# Autodesk Inventor assembly: launcher.mainAssembly
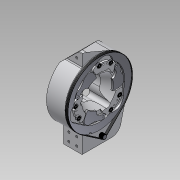
[picture p0: Inventor's stored thumbnail of the model, 180x180]
Saved by Autodesk Inventor 2011 (Build 150239000, 239)
## iProperties
Created: 2011-02-22
Part Number: launcher.mainAssembly
Document SubType Name: Assembly
Designer: Casey
Author: Casey
## Documents named in this file (8)
- C:\Users\Casey\Documents\My Dropbox\RockSAT-X 2011 RexSAT\capsule-launcher.design\Launcher\launcher.mainAssembly.iam
- C:\Users\Casey\Documents\My Dropbox\RockSAT-X 2011 RexSAT\capsule-launcher.design\Launcher\launcher.housing.ipt
- C:\Users\Casey\Documents\My Dropbox\RockSAT-X 2011 RexSAT\capsule-launcher.design\Capsule\capsule.final.assembly.iam
- C:\Users\Casey\Documents\My Dropbox\RockSAT-X 2011 RexSAT\capsule-launcher.design\Launcher\3x8x4_bearing.ipt
- C:\Users\Casey\Documents\My Dropbox\RockSAT-X 2011 RexSAT\capsule-launcher.design\Launcher\launcher.cap.ipt
- C:\Users\Casey\Documents\My Dropbox\RockSAT-X 2011 RexSAT\capsule-launcher.design\Launcher\launcher.cam.ipt
- C:\Users\Casey\Documents\My Dropbox\RockSAT-X 2011 RexSAT\capsule-launcher.design\Launcher\launcher.latch.ipt
- C:\Users\Casey\Documents\My Dropbox\RockSAT-X 2011 RexSAT\capsule-launcher.design\Launcher\launcher.mainAssembly\Design Accelerator\Synchronous Belts Transmission2.iam
## Components (17 placed, 7 different names)
1. launcher.housing:1 — Mate:7, Tangent:5, Mate:8, Mate:9, Mate:10, Mate:11, Mate:12, Mate:13, Flush:5, Mate:14, Mate:15, Mate:16, Flush:7, Mate:17, Mate:18, Mate:19, Mate:24, Mate:25, Mate:26
2. capsule.final.assembly:1 [sub-assembly] — Mate:7, Tangent:5
3. 3x8x4_bearing:1 — Mate:13, Flush:2, Flush:3
4. 3x8x4_bearing:2 — Mate:12, Flush:2, Flush:4
5. 3x8x4_bearing:3 — Mate:11, Flush:4, Flush:6
6. 3x8x4_bearing:4 — Mate:10, Flush:6
7. 3x8x4_bearing:5 — Mate:9, Flush:1, Flush:5
8. 3x8x4_bearing:6 — Mate:8, Flush:1, Flush:3
9. 3x8x4_bearing:7 — Mate:14, Flush:7, Flush:8
10. 3x8x4_bearing:8 — Mate:15, Flush:9
11. 3x8x4_bearing:9 — Mate:16, Flush:8, Flush:9, Mate:23
12. launcher.cap:1 — Mate:17, Mate:18, Mate:19
13. launcher.cam:1 — Mate:25, Mate:26
14. Synchronous Belts Transmission:1 [sub-assembly]
15. launcher.latch:1 — Mate:23, Mate:24
16. launcher.latch:2
17. launcher.latch:3
## Component patterns: (3 elements, first: launcher.latch:1)
## Relationships (27: Mate 17, Flush 9, Tangent 1)
- Mate:7: launcher.housing:1 ↔ capsule.final.assembly:1
- Tangent:5: launcher.housing:1 ↔ capsule.final.assembly:1
- Mate:8: launcher.housing:1 ↔ 3x8x4_bearing:6
- Mate:9: launcher.housing:1 ↔ 3x8x4_bearing:5
- Mate:10: launcher.housing:1 ↔ 3x8x4_bearing:4
- Mate:11: launcher.housing:1 ↔ 3x8x4_bearing:3
- Mate:12: launcher.housing:1 ↔ 3x8x4_bearing:2
- Mate:13: launcher.housing:1 ↔ 3x8x4_bearing:1
- Flush:1: 3x8x4_bearing:5 ↔ 3x8x4_bearing:6
- Flush:2: 3x8x4_bearing:1 ↔ 3x8x4_bearing:2
- Flush:3: 3x8x4_bearing:1 ↔ 3x8x4_bearing:6
- Flush:4: 3x8x4_bearing:2 ↔ 3x8x4_bearing:3
- Flush:5: launcher.housing:1 ↔ 3x8x4_bearing:5
- Flush:6: 3x8x4_bearing:3 ↔ 3x8x4_bearing:4
- Mate:14: launcher.housing:1 ↔ 3x8x4_bearing:7
- Mate:15: launcher.housing:1 ↔ 3x8x4_bearing:8
- Mate:16: launcher.housing:1 ↔ 3x8x4_bearing:9
- Flush:7: launcher.housing:1 ↔ 3x8x4_bearing:7
- Flush:8: 3x8x4_bearing:7 ↔ 3x8x4_bearing:9
- Flush:9: 3x8x4_bearing:8 ↔ 3x8x4_bearing:9
- Mate:17: launcher.housing:1 ↔ launcher.cap:1
- Mate:18: launcher.housing:1 ↔ launcher.cap:1
- Mate:19: launcher.housing:1 ↔ launcher.cap:1
- Mate:23: 3x8x4_bearing:9 ↔ launcher.latch:1
- Mate:24: launcher.housing:1 ↔ launcher.latch:1
- Mate:25: launcher.housing:1 ↔ launcher.cam:1
- Mate:26: launcher.housing:1 ↔ launcher.cam:1
